# Autodesk Inventor assembly: Ensemble1
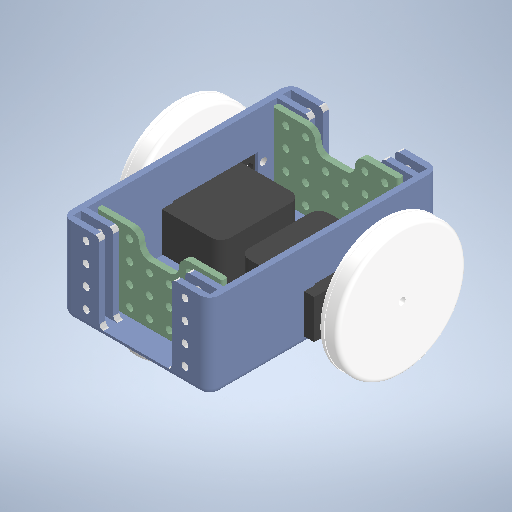
[picture p0: Inventor's stored thumbnail of the model, 512x512]
Saved by Autodesk Inventor 2025 (Build 290162000, 162)
## iProperties
Created: 2024-09-06
Part Number: Ensemble1
Document SubType Name: Assembly
Designer: chass
Author: chass
## Documents named in this file (5)
- C:\Users\chass\Documents\AREM\Hackathon_2024\Modeles_3D\Ensemble1.iam
- C:\Users\chass\Documents\AREM\Hackathon_2024\Modeles_3D\chassis.ipt
- C:\Users\chass\Documents\AREM\Hackathon_2024\Modeles_3D\servomoteur_roues.ipt
- C:\Users\chass\Documents\AREM\Hackathon_2024\Modeles_3D\roue.ipt
- C:\Users\chass\Documents\AREM\Hackathon_2024\Modeles_3D\plaque.ipt
## Components (7 placed, 4 different names)
1. chassis:1 — Placage:1, Placage:2, Placage:3, Placage:6, Placage:7, Placage:8, Placage:11, Placage:12, Placage:13, Placage:14, Placage:15, Placage:16
2. roue:1 — Placage:4, Placage:5
3. roue:2 — Placage:9, Placage:10
4. servomoteur_roues:1 — Placage:1, Placage:2, Placage:3, Placage:4, Placage:5
5. servomoteur_roues:2 — Placage:6, Placage:7, Placage:8, Placage:9, Placage:10
6. plaque:1 — Placage:11, Placage:12, Placage:13
7. plaque:2 — Placage:14, Placage:15, Placage:16
## Relationships (16: Mate 16)
- Placage:1 [Mate]: chassis:1 ↔ servomoteur_roues:1
- Placage:2 [Mate]: chassis:1 ↔ servomoteur_roues:1
- Placage:3 [Mate]: chassis:1 ↔ servomoteur_roues:1
- Placage:4 [Mate]: roue:1 ↔ servomoteur_roues:1
- Placage:5 [Mate]: roue:1 ↔ servomoteur_roues:1
- Placage:6 [Mate]: chassis:1 ↔ servomoteur_roues:2
- Placage:7 [Mate]: chassis:1 ↔ servomoteur_roues:2
- Placage:8 [Mate]: chassis:1 ↔ servomoteur_roues:2
- Placage:9 [Mate]: roue:2 ↔ servomoteur_roues:2
- Placage:10 [Mate]: roue:2 ↔ servomoteur_roues:2
- Placage:11 [Mate]: chassis:1 ↔ plaque:1
- Placage:12 [Mate]: chassis:1 ↔ plaque:1
- Placage:13 [Mate]: chassis:1 ↔ plaque:1
- Placage:14 [Mate]: chassis:1 ↔ plaque:2
- Placage:15 [Mate]: chassis:1 ↔ plaque:2
- Placage:16 [Mate]: chassis:1 ↔ plaque:2
